# Autodesk Inventor assembly: ORBITS Frame
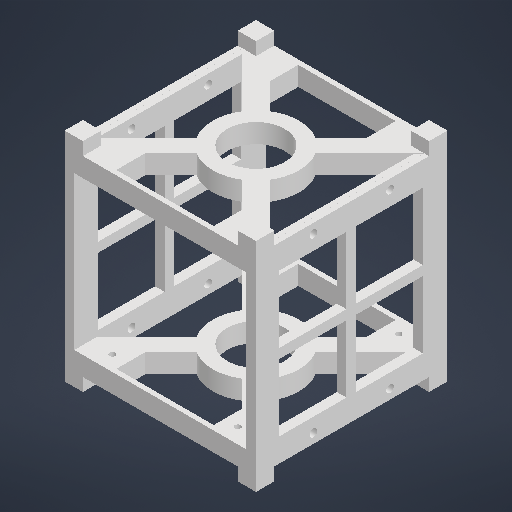
[picture p0: Inventor's stored thumbnail of the model, 512x512]
Saved by Autodesk Inventor 2026.1 (Build 301233020, 233B)
## iProperties
Created: 2025-10-16
Part Number: ORBITS Frame
Document SubType Name: Assembly
Designer: scott
Author: scott
## Documents named in this file (3)
- C:\Users\Public\Documents\Autodesk\Inventor 2026\EE475\ORBITS Frame.iam
- C:\Users\Public\Documents\Autodesk\Inventor 2026\EE475\Top&Bottom.ipt
- C:\Users\Public\Documents\Autodesk\Inventor 2026\EE475\Side Panel.ipt
## Components (4 placed, 2 different names)
1. Top&Bottom:1 — Angle:1, Flush:1, Mate:5, Mate:6
2. Top&Bottom:2 — Angle:1, Flush:1, Mate:1, Mate:2, Mate:3, Mate:4
3. Side Panel:1 — Mate:3, Mate:4
4. Side Panel:2 — Mate:1, Mate:2, Mate:5, Mate:6
## Relationships (8: Mate 6, Angle 1, Flush 1)
- Angle:1 (180 deg): Top&Bottom:1 ↔ Top&Bottom:2
- Flush:1: Top&Bottom:1 ↔ Top&Bottom:2
- Mate:1: Top&Bottom:2 ↔ Side Panel:2
- Mate:2: Top&Bottom:2 ↔ Side Panel:2
- Mate:3: Top&Bottom:2 ↔ Side Panel:1
- Mate:4: Top&Bottom:2 ↔ Side Panel:1
- Mate:5: Top&Bottom:1 ↔ Side Panel:2
- Mate:6: Top&Bottom:1 ↔ Side Panel:2
